# Autodesk Inventor assembly: check_end_assembly
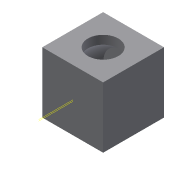
[picture p0: Inventor's stored thumbnail of the model, 180x180]
Saved by Autodesk Inventor 2017 (Build 210142000, 142)
## iProperties
Created: 2018-07-07
Part Number: check_end_assembly
Document SubType Name: Assembly
Designer: Nic
Author: Nic
## Documents named in this file (4)
- C:\Users\Nic\Documents\Antenna\check_end_assembly.iam
- C:\Users\Nic\Documents\Antenna\mould_end_casing_base_v3.ipt
- C:\Users\Nic\Documents\Antenna\mould_end_casing_top_v3.ipt
- C:\Users\Nic\Documents\Antenna\end_segment_v3.ipt
## Components (3 placed, 3 different names)
1. mould_end_casing_base_v3:1 — Flush:1, Insert:2
2. mould_end_casing_top_v3:1 — Insert:1, Flush:1, Insert:2
3. end_segment_v3:1 — Insert:1
## Relationships (3: Insert 2, Flush 1)
- Insert:1 (0.2 mm): mould_end_casing_top_v3:1 ↔ end_segment_v3:1
- Flush:1: mould_end_casing_base_v3:1 ↔ mould_end_casing_top_v3:1
- Insert:2: mould_end_casing_base_v3:1 ↔ mould_end_casing_top_v3:1
